# Autodesk Inventor assembly: sb_lid_assembly
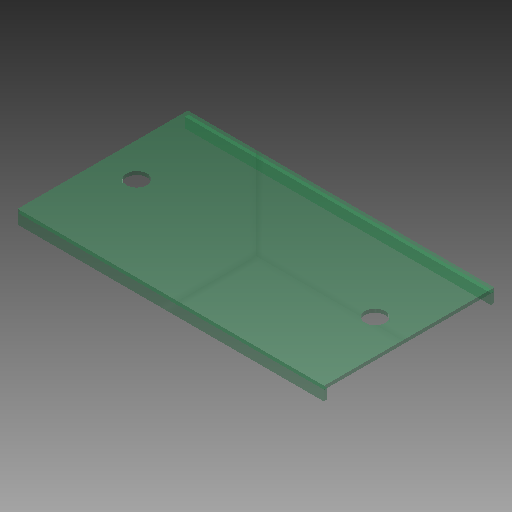
[picture p0: Inventor's stored thumbnail of the model, 512x512]
Saved by Autodesk Inventor 2018.1 (Build 221171000, 171)
## iProperties
Created: 2017-08-17
Part Number: sb_lid_assembly
Document SubType Name: Assembly
Designer: Tom
Author: Tom
## Documents named in this file (4)
- \\Mac\Dropbox\2015-2016\Bachelorproef\Inventor\Electronics and Solenoids Box\eb_separator_assembly.iam
- \\Mac\Dropbox\2015-2016\Bachelorproef\Inventor\Electronics and Solenoids Box\eb_separator.ipt
- \\Mac\Dropbox\2015-2016\Bachelorproef\Inventor\Electronics and Solenoids Box\eb_separator_support.ipt
- \\Mac\Dropbox\2015-2016\Bachelorproef\Inventor\Electronics and Solenoids Box\par_sol_box.xls
## Components (3 placed, 2 different names)
1. eb_separator:1 — Mate:1, Mate:2, Flush:1, Flush:2, Flush:3, Flush:4
2. eb_separator_support:1 — Mate:1, Flush:2, Flush:3
3. eb_separator_support:2 — Mate:2, Flush:1, Flush:4
## Relationships (6: Flush 4, Mate 2)
- Mate:1: eb_separator:1 ↔ eb_separator_support:1
- Mate:2: eb_separator:1 ↔ eb_separator_support:2
- Flush:1: eb_separator:1 ↔ eb_separator_support:2
- Flush:2: eb_separator:1 ↔ eb_separator_support:1
- Flush:3 (0.5 mm): eb_separator:1 ↔ eb_separator_support:1
- Flush:4 (0.5 mm): eb_separator:1 ↔ eb_separator_support:2
## Named parameters: solhole = 3 mm, solholespacing = 16 mm, ssoll = 70 mm, ssolw = 63 mm, bsoll = 126 mm, bsolw = 91 mm, bsolh = 126 mm, tapl = 31 mm, tl = 32 mm, tw = 50 mm, eloboww = 25 mm, pvct = 5 mm, boxw = 450 mm, boxl = 250 mm, boxh = 258 mm, supporth = 15 mm, play = 0.5 mm, sidedist = 90 mm, pcbw = 76 mm, pcbh = 46 mm, psul = 140 mm, screenl = 115 mm, screent = 50 mm, psuw = 150 mm, pcbl = 86 mm, arl = 102 mm, psuh = 85 mm, arw = 54 mm, screenw = 197 mm, seph = 105 mm, dialoadouter = 25 mm, diaetapeouter = 36 mm, diaload = 16 mm, diaetape = 25 mm, diaph = 32 mm, diaphouter = 48 mm, diapowerouter = 25 mm, diapower = 16 mm, distsidepump = 120 mm, waterinner = 28 mm, distpumpbubble = 100 mm, distpumps = 75 mm, waterouter = 39 mm, airoutinner = 28 mm, pumpouter = 25 mm, distbubblewater = 82 mm, pumpinner = 16 mm, airininner = 28 mm, airinouter = 39 mm, airoutouter = 39 mm, distsidewater = 100 mm
